# Autodesk Inventor assembly: Kegelrad
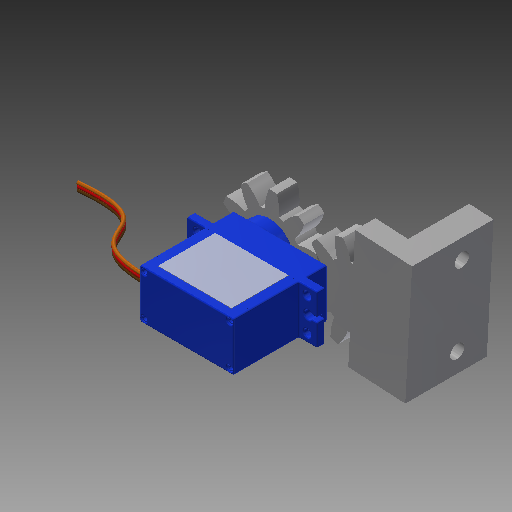
[picture p0: Inventor's stored thumbnail of the model, 512x512]
Saved by Autodesk Inventor 2018 (Build 220112000, 112)
## iProperties
Created: 2018-01-26
Part Number: Kegelrad
Material: Generisch
Document SubType Name: Assembly
Designer: gchri
Author: gchri
## Documents named in this file (3)
- C:\Users\gchri\OneDrive\Development\RTW\03_Konstruktion\StirnradUNDServo.iam
- C:\Users\gchri\Downloads\Servo HXT900 Micro.iam
- C:\Users\gchri\OneDrive\Development\RTW\03_Konstruktion\StirnradUNDServo\Konstruktions-Assistent\Stirnräder1.iam
## Components (2 placed, 2 different names)
1. Servo HXT900 Micro:1 [sub-assembly] — Passend:1, Passend:2
2. Stirnräder:1 [sub-assembly] — Passend:1, Passend:2
## Relationships (2: Mate 2)
- Passend:1 [Mate]: Servo HXT900 Micro:1 ↔ Stirnräder:1
- Passend:2 [Mate]: Servo HXT900 Micro:1 ↔ Stirnräder:1
